# Autodesk Inventor assembly: lazysusan
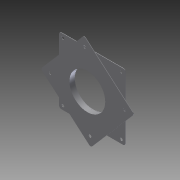
[picture p0: Inventor's stored thumbnail of the model, 180x180]
Saved by Autodesk Inventor 2011 (Build 150239000, 239)
## iProperties
Created: 2011-09-17
Part Number: lazysusan
Document SubType Name: Assembly
Designer: Matthew
Author: Matthew
## Documents named in this file (3)
- C:\Users\Matthew\Documents\matthew_autocad\prlite\lazy susan\lazysusan.iam
- C:\Users\Matthew\Documents\matthew_autocad\prlite\lazy susan\1.ipt
- C:\Users\Matthew\Documents\matthew_autocad\prlite\lazy susan\2.ipt
## Components (2 placed, 2 different names)
1. 1:1 — Mate:1, Mate:2
2. 2:1 — Mate:1, Mate:2
## Relationships (2: Mate 2)
- Mate:1: 1:1 ↔ 2:1
- Mate:2: 1:1 ↔ 2:1
